# Autodesk Inventor assembly: PitchAssemblyNFinal
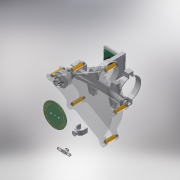
[picture p0: Inventor's stored thumbnail of the model, 180x180]
Saved by Autodesk Inventor 2018.2 (Build 222227000, 227)
## iProperties
Created: 2018-04-02
Part Number: PitchAssemblyNFinal
Document SubType Name: Assembly
Designer: Muchen He
Author: Muchen He
## Documents named in this file (17)
- C:\Users\Moochster\OneDrive\Documents\2018 UBC\ELEC 391\Controller\cad\release\PitchAssemblyNFinal.iam
- C:\Users\Moochster\OneDrive\Documents\2018 UBC\ELEC 391\Controller\cad\release\RailBase.ipt
- C:\Users\Moochster\OneDrive\Documents\2018 UBC\ELEC 391\Controller\cad\release\RailBaseBottom.ipt
- C:\Users\Moochster\OneDrive\Documents\2018 UBC\ELEC 391\Controller\cad\release\Fasteners\StandoffM4x20B.ipt
- C:\Users\Moochster\OneDrive\Documents\2018 UBC\ELEC 391\Controller\cad\release\R1038_ZZ_W Bearing.ipt
- C:\Users\Moochster\OneDrive\Documents\2018 UBC\ELEC 391\Controller\cad\release\Rod3_8in.ipt
- C:\Users\Moochster\OneDrive\Documents\2018 UBC\ELEC 391\Controller\cad\release\ShaftArm.ipt
- C:\Users\Moochster\OneDrive\Documents\2018 UBC\ELEC 391\Controller\cad\release\ShaftBushing.ipt
- C:\Users\Moochster\OneDrive\Documents\2018 UBC\ELEC 391\Controller\cad\release\ShaftSyncAdapter.ipt
- C:\Users\Moochster\OneDrive\Documents\2018 UBC\ELEC 391\Controller\cad\release\OmegaRing.ipt
- C:\Users\Moochster\OneDrive\Documents\2018 UBC\ELEC 391\Controller\cad\release\OmegaRingTypeC.ipt
- C:\Users\Moochster\OneDrive\Documents\2018 UBC\ELEC 391\Controller\cad\release\EncoderPCBAssembly.iam
- C:\Users\Moochster\OneDrive\Documents\2018 UBC\ELEC 391\Controller\cad\release\EncoderWheelAdapterSmallSlotted.ipt
- C:\Users\Moochster\OneDrive\Documents\2018 UBC\ELEC 391\Controller\cad\release\EncoderWheelPitch.ipt
- C:\Users\Moochster\OneDrive\Documents\2018 UBC\ELEC 391\Controller\cad\release\GT2TimingBeltGear.ipt
- C:\Users\Moochster\OneDrive\Documents\2018 UBC\ELEC 391\Controller\cad\release\LaserDiodeAdapterLarge.ipt
- C:\Users\Moochster\OneDrive\Documents\2018 UBC\ELEC 391\Controller\cad\release\SecondaryEncoderPCBMount.ipt
## Components (23 placed, 16 different names)
1. RailBase:1 — Mate:1, Insert:7, Insert:8
2. RailBaseBottom:1 — Mate:1, Insert:1, Insert:2, Insert:3, Insert:4, Insert:5, Insert:6, Mate:2, Insert:9, Mate:18
3. StandoffM4x20B:1 — Insert:6
4. StandoffM4x20B:2 — Insert:5, Insert:7
5. StandoffM4x20B:3 — Insert:4
6. StandoffM4x20B:4 — Insert:3
7. StandoffM4x20B:5 — Insert:2
8. StandoffM4x20B:6 — Insert:1
9. R1038_ZZ_W Bearing:1 — Insert:9
10. R1038_ZZ_W Bearing:2 — Insert:8, Mate:16
11. R1038_ZZ_W Bearing:3 — Insert:10
12. Rod3_8in:1 — Mate:2, Mate:3, Mate:4, Mate:5, Mate:10
13. ShaftArm:1 — Mate:3, Mate:6, Mate:7, Mate:8, Mate:9, Insert:10, Mate:13, Mate:14, Mate:15, Mate:17
14. ShaftBushing:1 — Mate:4, Mate:16, Mate:17
15. ShaftSyncAdapter:1 — Mate:5, Mate:15
16. OmegaRing:1 — Mate:8, Mate:9, Insert:11, Insert:12, Mate:13
17. OmegaRingTypeC:1 — Mate:6, Mate:7, Mate:14
18. EncoderPCBAssembly:1 [sub-assembly] — Mate:11, Mate:12, Mate:19
19. EncoderWheelAdapterSmallSlotted:1
20. EncoderWheelPitch:1
21. GT2TimingBeltGear:1 — Mate:10, Mate:18
22. LaserDiodeAdapterLarge:1
23. SecondaryEncoderPCBMount:1 — Insert:11, Insert:12, Mate:11, Mate:12, Mate:19
## Relationships (31: Mate 19, Insert 12)
- Mate:1: RailBase:1 ↔ RailBaseBottom:1
- Insert:1: RailBaseBottom:1 ↔ StandoffM4x20B:6
- Insert:2: RailBaseBottom:1 ↔ StandoffM4x20B:5
- Insert:3: RailBaseBottom:1 ↔ StandoffM4x20B:4
- Insert:4: RailBaseBottom:1 ↔ StandoffM4x20B:3
- Insert:5: RailBaseBottom:1 ↔ StandoffM4x20B:2
- Insert:6: RailBaseBottom:1 ↔ StandoffM4x20B:1
- Insert:7: RailBase:1 ↔ StandoffM4x20B:2
- Mate:2: RailBaseBottom:1 ↔ Rod3_8in:1
- Insert:8: RailBase:1 ↔ R1038_ZZ_W Bearing:2
- Insert:9: RailBaseBottom:1 ↔ R1038_ZZ_W Bearing:1
- Mate:3: Rod3_8in:1 ↔ ShaftArm:1
- Mate:4: Rod3_8in:1 ↔ ShaftBushing:1
- Mate:5: Rod3_8in:1 ↔ ShaftSyncAdapter:1
- Mate:6: ShaftArm:1 ↔ OmegaRingTypeC:1
- Mate:7: ShaftArm:1 ↔ OmegaRingTypeC:1
- Mate:8: ShaftArm:1 ↔ OmegaRing:1
- Mate:9: ShaftArm:1 ↔ OmegaRing:1
- Insert:10: R1038_ZZ_W Bearing:3 ↔ ShaftArm:1
- Mate:10: Rod3_8in:1 ↔ GT2TimingBeltGear:1
- Insert:11: OmegaRing:1 ↔ SecondaryEncoderPCBMount:1
- Insert:12: OmegaRing:1 ↔ SecondaryEncoderPCBMount:1
- Mate:11: EncoderPCBAssembly:1 ↔ SecondaryEncoderPCBMount:1
- Mate:12: EncoderPCBAssembly:1 ↔ SecondaryEncoderPCBMount:1
- Mate:13 (0.1 mm): ShaftArm:1 ↔ OmegaRing:1
- Mate:14 (0.1 mm): ShaftArm:1 ↔ OmegaRingTypeC:1
- Mate:15: ShaftArm:1 ↔ ShaftSyncAdapter:1
- Mate:16 (0.1 mm): R1038_ZZ_W Bearing:2 ↔ ShaftBushing:1
- Mate:17 (0.1 mm): ShaftArm:1 ↔ ShaftBushing:1
- Mate:18 (1 mm): RailBaseBottom:1 ↔ GT2TimingBeltGear:1
- Mate:19 (2 mm): EncoderPCBAssembly:1 ↔ SecondaryEncoderPCBMount:1
